# Autodesk Inventor assembly: Cable Poder 220V
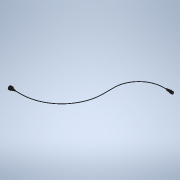
[picture p0: Inventor's stored thumbnail of the model, 180x180]
Saved by Autodesk Inventor 2020.3 (Build 243373000, 373)
## iProperties
Created: 2020-07-06
Part Number: Cable Poder 220V
Document SubType Name: Assembly
Designer: Bruno
Author: Bruno
## Documents named in this file (4)
- C:\Users\Bruno\Desktop\Cable 220V\Cable Poder 220V.iam
- C:\Users\Bruno\Desktop\Cable 220V\IEC 320 C13 Cable End.ipt
- C:\Users\Bruno\Desktop\Cable 220V\Cable 220V - 2.5in - 1.5m.ipt
- C:\Users\Bruno\Desktop\Cable 220V\AC plug.ipt
## Components (3 placed, 3 different names)
1. IEC 320 C13 Cable End:1 — Flush:1, Flush:3
2. Cable 220V - 2.5in - 1.5m:1 — Flush:1, Flush:3, Cylindrical:1
3. AC plug:1 — Cylindrical:1
## Relationships (3: Flush 2, CylindricalJoint 1)
- Flush:1: IEC 320 C13 Cable End:1 ↔ Cable 220V - 2.5in - 1.5m:1
- Flush:3: IEC 320 C13 Cable End:1 ↔ Cable 220V - 2.5in - 1.5m:1
- Cylindrical:1: Cable 220V - 2.5in - 1.5m:1 ↔ AC plug:1
